# Autodesk Inventor assembly: Coluna_Suspensao_4-Cabos_Modelo1
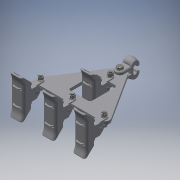
[picture p0: Inventor's stored thumbnail of the model, 180x180]
Saved by Autodesk Inventor 2018 (Build 220112000, 112)
## iProperties
Created: 2021-08-02
Part Number: Coluna_Suspensao_4-Cabos_Modelo1
Document SubType Name: Assembly
Designer: L08619
Author: L08619
## Documents named in this file (4)
- C:\Users\l08619\Documents\Projetos\TAESA\Modelo 3D - Tensionadores e Suspensão\Suporte de Suspenção\Coluna_Suspensao_4-Cabos_Modelo1.iam
- C:\Users\l08619\Documents\Projetos\TAESA\Modelo 3D - Tensionadores e Suspensão\Suporte de Suspenção\Corpo_Suporte_4_Cabos_Modelo1.ipt
- C:\Users\l08619\Documents\Projetos\TAESA\Modelo 3D - Tensionadores e Suspensão\Suporte de Suspenção\Suspenssion_Clamp.iam
- C:\Users\l08619\Documents\Projetos\TAESA\Modelo 3D - Tensionadores e Suspensão\Suporte de Suspenção\Clevis-Socket.iam
## Components (6 placed, 3 different names)
1. Corpo_Suporte_4_Cabos_Modelo1:1 — Mate:1, Mate:2, Cylindrical:1, Cylindrical:2, Cylindrical:3, Cylindrical:4, Cylindrical:5, Mate:3, Mate:4, Mate:5, Mate:6, Mate:7
2. Suspenssion_Clamp:1 [sub-assembly] — Cylindrical:3, Mate:4
3. Suspenssion_Clamp:2 [sub-assembly] — Cylindrical:2, Mate:7
4. Suspenssion_Clamp:3 [sub-assembly] — Cylindrical:5, Mate:6
5. Suspenssion_Clamp:4 [sub-assembly] — Cylindrical:4, Mate:5
6. Clevis-Socket:1 [sub-assembly] — Cylindrical:1, Mate:3
## Relationships (12: Mate 7, CylindricalJoint 5)
- Mate:1: Corpo_Suporte_4_Cabos_Modelo1:1
- Mate:2: Corpo_Suporte_4_Cabos_Modelo1:1
- Cylindrical:1: Corpo_Suporte_4_Cabos_Modelo1:1 ↔ Clevis-Socket:1
- Cylindrical:2: Corpo_Suporte_4_Cabos_Modelo1:1 ↔ Suspenssion_Clamp:2
- Cylindrical:3: Corpo_Suporte_4_Cabos_Modelo1:1 ↔ Suspenssion_Clamp:1
- Cylindrical:4: Corpo_Suporte_4_Cabos_Modelo1:1 ↔ Suspenssion_Clamp:4
- Cylindrical:5: Corpo_Suporte_4_Cabos_Modelo1:1 ↔ Suspenssion_Clamp:3
- Mate:3 (3 mm): Corpo_Suporte_4_Cabos_Modelo1:1 ↔ Clevis-Socket:1
- Mate:4 (3 mm): Corpo_Suporte_4_Cabos_Modelo1:1 ↔ Suspenssion_Clamp:1
- Mate:5 (3 mm): Corpo_Suporte_4_Cabos_Modelo1:1 ↔ Suspenssion_Clamp:4
- Mate:6 (3 mm): Corpo_Suporte_4_Cabos_Modelo1:1 ↔ Suspenssion_Clamp:3
- Mate:7 (3 mm): Corpo_Suporte_4_Cabos_Modelo1:1 ↔ Suspenssion_Clamp:2
